# Autodesk Inventor assembly: RouveV4
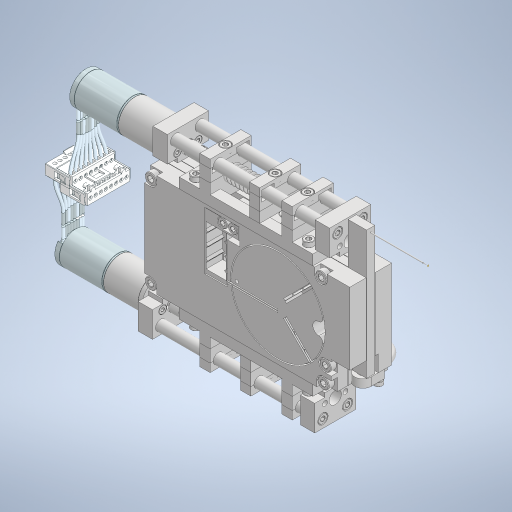
[picture p0: Inventor's stored thumbnail of the model, 512x512]
Saved by Autodesk Inventor 2023 (Build 270158000, 158)
## iProperties
Created: 2023-05-10
Part Number: RouveV4
Document SubType Name: Assembly
Designer: Nathann
Author: Nathann
## Documents named in this file (27)
- C:\Users\Nathann\OneDrive\ClawdDrive\Objet3D\IminaProbe\V4Roue\RouveV4.iam
- C:\Users\Nathann\OneDrive\ClawdDrive\Objet3D\IminaProbe\V4Roue\4145N198_Set Screw Precision Flexible Shaft Couplings.ipt
- C:\Users\Nathann\OneDrive\ClawdDrive\Objet3D\IminaProbe\V4Roue\283825_ec-max16_5w.ipt
- C:\Users\Nathann\OneDrive\ClawdDrive\Objet3D\IminaProbe\V4Roue\AngleScrewBlocActuator.ipt
- C:\Users\Nathann\OneDrive\ClawdDrive\Objet3D\IminaProbe\V4Roue\AxisLinear.ipt
- C:\Users\Nathann\OneDrive\ClawdDrive\Objet3D\IminaProbe\V4Roue\CapacitiveSensor.ipt
- C:\Users\Nathann\OneDrive\ClawdDrive\Objet3D\IminaProbe\V4Roue\MotorDifferentialMountingBracket.ipt
- C:\Users\Nathann\OneDrive\ClawdDrive\Objet3D\IminaProbe\V4Roue\MotorMountDifferential.ipt
- C:\Users\Nathann\OneDrive\ClawdDrive\Objet3D\IminaProbe\V4Roue\POMSliderAxis.ipt
- C:\Users\Nathann\OneDrive\ClawdDrive\Objet3D\IminaProbe\V4Roue\POMSliderMotor.ipt
- C:\Users\Nathann\OneDrive\ClawdDrive\Objet3D\IminaProbe\V4Roue\POMSliderMotorM25.ipt
- C:\Users\Nathann\OneDrive\ClawdDrive\Objet3D\IminaProbe\V4Roue\Probe.ipt
- C:\Users\Nathann\OneDrive\ClawdDrive\Objet3D\IminaProbe\V4Roue\RoueV3partA.ipt
- C:\Users\Nathann\OneDrive\ClawdDrive\Objet3D\IminaProbe\V4Roue\RoueV3PartB.ipt
- C:\Users\Nathann\OneDrive\ClawdDrive\Objet3D\IminaProbe\V4Roue\RoueV3PartC.ipt
- C:\Users\Nathann\OneDrive\ClawdDrive\Objet3D\IminaProbe\V4Roue\SliderFixtureM25.ipt
- C:\Users\Nathann\OneDrive\ClawdDrive\Objet3D\IminaProbe\V4Roue\Sprint.ipt
- C:\Users\Nathann\OneDrive\ClawdDrive\Objet3D\IminaProbe\V4Roue\GP16A_2-Stufig-110322.ipt
- C:\Users\Nathann\OneDrive\ClawdDrive\Objet3D\IminaProbe\V4Roue\Screw.ipt
- C:\Users\Nathann\ClawdDrive\Objet3D\IminaProbe\V3Roue\91292A009_18-8 Stainless Steel Socket Head Screw.ipt
- C:\Users\Nathann\ClawdDrive\Objet3D\IminaProbe\V3Roue\91292A832_18-8 Stainless Steel Socket Head Screw.ipt
- C:\Users\Nathann\ClawdDrive\Objet3D\IminaProbe\V3Roue\91828A113_18-8 Stainless Steel Hex Nut.ipt
- C:\Users\Nathann\ClawdDrive\Objet3D\IminaProbe\V3Roue\91828A211_18-8 Stainless Steel Hex Nut.ipt
- C:\Users\Nathann\OneDrive\ClawdDrive\Objet3D\IminaProbe\V4Roue\91292A012_18-8 Stainless Steel Socket Head Screw.ipt
- C:\Users\Nathann\OneDrive\ClawdDrive\Objet3D\IminaProbe\V4Roue\91292A114_18-8 Stainless Steel Socket Head Screw.ipt
- C:\Users\Nathann\OneDrive\ClawdDrive\Objet3D\IminaProbe\V4Roue\clinquantSpacer.ipt
- C:\Users\Nathann\OneDrive\ClawdDrive\Objet3D\IminaProbe\V4Roue\boundingBox.ipt
## Components (105 placed, 26 different names)
1. 4145N198_Set Screw Precision Flexible Shaft Couplings:1 — Insert:12, Insert:46
2. 283825_ec-max16_5w:1 — Insert:1, Mate:135
3. AngleScrewBlocActuator:1 — Insert:47, Insert:48
4. AxisLinear:1 — Mate:59, Mate:60, Insert:4, Insert:6, Mate:131
5. CapacitiveSensor:1 — Mate:2, Flush:7, Mate:3, Mate:4, Mate:37, Mate:38, Mate:39
6. MotorDifferentialMountingBracket:1 — Mate:47, Mate:48, Mate:49, Mate:50, Flush:12, Flush:13, Flush:14, Flush:15, Mate:51, Mate:52, Mate:53, Mate:54, Mate:55, Mate:56, Mate:57, Mate:58, Mate:73, Mate:75, Flush:25, Flush:26, Mate:118, Mate:119, Mate:120, Mate:121, Mate:122, Insert:31, Insert:32, Insert:33, Insert:34, Flush:42, Flush:45
7. MotorMountDifferential:1 — Mate:59, Mate:62, Mate:63, Mate:64, Mate:65, Mate:66, Mate:69, Mate:70, Insert:6, Insert:7, Insert:8, Insert:9, Insert:10, Insert:11
8. POMSliderAxis:1 — Flush:35, Flush:40, Mate:113, Mate:124, Insert:39
9. POMSliderMotor:1 — Flush:12, Flush:14, Mate:57, Flush:32, Mate:125, Mate:130
10. POMSliderMotorM25:1 — Flush:9, Flush:10, Mate:44, Mate:45, Mate:46, Flush:30, Flush:33, Mate:126, Flush:45
11. Probe:1 — Mate:1, Flush:8
12. RoueV3partA:1 — Flush:5, Flush:6, Mate:2, Flush:7, Mate:15, Mate:16, Mate:17, Mate:18, Mate:19, Mate:30, Mate:37, Angle:1, Mate:122, Mate:123
13. RoueV3PartB:1 — Flush:2, Flush:4, Mate:1, Flush:5, Flush:6, Mate:10, Mate:11, Mate:12, Mate:13, Mate:14, Mate:20, Mate:21, Mate:22, Mate:23, Mate:24, Mate:25, Mate:26, Mate:27, Mate:28, Mate:29, Flush:8
14. RoueV3PartC:1 — Flush:2, Flush:4, Mate:5, Mate:6, Mate:7, Mate:8, Mate:9, Mate:31, Mate:32, Mate:33, Mate:34, Mate:35, Mate:36, Flush:25, Flush:28, Flush:41, Mate:133, Mate:134, Insert:49, Insert:50, Mate:135
15. SliderFixtureM25:1 — Flush:9, Flush:10, Flush:11, Mate:45, Insert:2, Insert:3, Mate:73, Insert:13, Insert:14, Insert:47, Insert:48
16. Sprint:1 — Mate:75
17. GP16A_2-Stufig-110322:1 — Insert:1, Mate:63, Mate:66, Insert:11, Insert:45
18. Screw:1 — Insert:12
19. 91292A009_18-8 Stainless Steel Socket Head Screw:1 — Mate:113, Insert:39
20. 91292A832_18-8 Stainless Steel Socket Head Screw:2 — Mate:64, Insert:10
21. 91828A113_18-8 Stainless Steel Hex Nut:2 — Flush:11, Mate:44, Mate:46
22. 91828A211_18-8 Stainless Steel Hex Nut:1 — Mate:55, Mate:56
23. 91292A114_18-8 Stainless Steel Socket Head Screw:1 — Mate:5, Mate:33
24. 91292A832_18-8 Stainless Steel Socket Head Screw:3 — Mate:4, Mate:39
25. 91292A832_18-8 Stainless Steel Socket Head Screw:4 — Mate:3, Mate:38
26. 91292A114_18-8 Stainless Steel Socket Head Screw:2 — Mate:6, Mate:32
27. 91292A114_18-8 Stainless Steel Socket Head Screw:3 — Mate:8, Mate:34
28. 91292A114_18-8 Stainless Steel Socket Head Screw:4 — Mate:9, Mate:35
29. 91292A114_18-8 Stainless Steel Socket Head Screw:5 — Mate:7, Mate:36
30. clinquantSpacer:1 — Mate:13, Mate:26
31. clinquantSpacer:2 — Mate:12, Mate:25, Mate:31
32. clinquantSpacer:3 — Mate:14, Mate:28
33. clinquantSpacer:4 — Mate:10, Mate:27
34. clinquantSpacer:5 — Mate:11, Mate:29
35. clinquantSpacer:6 — Mate:18, Mate:22, Mate:30
36. clinquantSpacer:7 — Mate:19, Mate:23
37. clinquantSpacer:8 — Mate:17, Mate:20
38. clinquantSpacer:9 — Mate:16, Mate:24
39. clinquantSpacer:10 — Mate:15, Mate:21
40. MotorMountDifferential:2 — Mate:60, Mate:61, Mate:67, Mate:68, Insert:4, Insert:5, Mate:71, Mate:72, Flush:27
41. POMSliderAxis:2 — Mate:107, Flush:37, Flush:38, Mate:129, Insert:41
42. POMSliderAxis:3 — Mate:108, Mate:128, Insert:40, Flush:43, Flush:44
43. POMSliderMotor:2 — Flush:13, Flush:15, Mate:58, Flush:34, Mate:127
44. AxisLinear:2 — Mate:61, Mate:62, Insert:5
45. 91292A012_18-8 Stainless Steel Socket Head Screw:3 — Mate:69, Insert:8
46. 91292A009_18-8 Stainless Steel Socket Head Screw:2 — Insert:2
47. 91292A009_18-8 Stainless Steel Socket Head Screw:3 — Insert:3
48. 91292A009_18-8 Stainless Steel Socket Head Screw:4 — Mate:48, Mate:53
49. 91292A009_18-8 Stainless Steel Socket Head Screw:5 — Mate:50, Mate:51
50. 91292A009_18-8 Stainless Steel Socket Head Screw:6 — Mate:47, Mate:52
51. 91292A009_18-8 Stainless Steel Socket Head Screw:7 — Mate:49, Mate:54
52. 91292A012_18-8 Stainless Steel Socket Head Screw:4 — Mate:70, Insert:7
53. 91292A012_18-8 Stainless Steel Socket Head Screw:5 — Mate:67, Mate:72
54. 91292A012_18-8 Stainless Steel Socket Head Screw:6 — Mate:68, Mate:71
55. 91292A832_18-8 Stainless Steel Socket Head Screw:5 — Mate:65, Insert:9
56. 91292A012_18-8 Stainless Steel Socket Head Screw:7 — Insert:14
57. 91292A012_18-8 Stainless Steel Socket Head Screw:8 — Insert:13
58. 4145N198_Set Screw Precision Flexible Shaft Couplings:2 — Insert:45
59. MotorDifferentialMountingBracket:2 — Flush:27, Flush:28, Mate:114, Mate:115, Mate:116, Mate:117, Angle:1, Mate:123, Insert:35, Insert:36, Insert:37, Insert:38, Flush:42, Mate:132
60. POMSliderMotor:3 — Flush:35, Flush:40, Mate:124, Mate:131
61. POMSliderMotorM25:2 — Mate:128, Flush:43, Flush:44
62. SliderFixtureM25:2 — Mate:132
63. Screw:2
64. 91828A113_18-8 Stainless Steel Hex Nut:3
65. 91828A211_18-8 Stainless Steel Hex Nut:2
66. POMSliderMotor:4 — Flush:37, Flush:38, Mate:129
67. 91292A009_18-8 Stainless Steel Socket Head Screw:8
68. 91292A009_18-8 Stainless Steel Socket Head Screw:9
69. 91292A009_18-8 Stainless Steel Socket Head Screw:10
70. 91292A009_18-8 Stainless Steel Socket Head Screw:11
71. 91292A009_18-8 Stainless Steel Socket Head Screw:12
72. 91292A009_18-8 Stainless Steel Socket Head Screw:13
73. 91292A012_18-8 Stainless Steel Socket Head Screw:9
74. 91292A012_18-8 Stainless Steel Socket Head Screw:10
75. 283825_ec-max16_5w:2
76. AxisLinear:3 — Mate:130
77. MotorMountDifferential:3 — Flush:41
78. GP16A_2-Stufig-110322:2 — Insert:46
79. 91292A832_18-8 Stainless Steel Socket Head Screw:6
80. MotorMountDifferential:4 — Flush:26
81. AxisLinear:4
82. 91292A012_18-8 Stainless Steel Socket Head Screw:11
83. 91292A012_18-8 Stainless Steel Socket Head Screw:12
84. 91292A012_18-8 Stainless Steel Socket Head Screw:13
85. 91292A012_18-8 Stainless Steel Socket Head Screw:14
86. 91292A832_18-8 Stainless Steel Socket Head Screw:7
87. POMSliderAxis:4 — Mate:112, Flush:32, Mate:125, Insert:42
88. POMSliderAxis:5 — Mate:110, Flush:34, Mate:127, Insert:44
89. POMSliderAxis:6 — Mate:111, Flush:30, Flush:33, Mate:126, Insert:43
90. 91292A009_18-8 Stainless Steel Socket Head Screw:14 — Mate:108, Insert:40
91. 91292A009_18-8 Stainless Steel Socket Head Screw:15 — Mate:107, Insert:41
92. 91292A009_18-8 Stainless Steel Socket Head Screw:16 — Mate:112, Insert:42
93. 91292A009_18-8 Stainless Steel Socket Head Screw:17 — Mate:111, Insert:43
94. 91292A009_18-8 Stainless Steel Socket Head Screw:18 — Mate:110, Insert:44
95. 91292A012_18-8 Stainless Steel Socket Head Screw:15 — Mate:114, Insert:36
96. 91292A012_18-8 Stainless Steel Socket Head Screw:16 — Mate:115, Insert:37
97. 91292A012_18-8 Stainless Steel Socket Head Screw:17 — Mate:117, Insert:38
98. 91292A012_18-8 Stainless Steel Socket Head Screw:18 — Mate:116, Insert:35
99. 91292A012_18-8 Stainless Steel Socket Head Screw:19 — Mate:121, Insert:34
100. 91292A012_18-8 Stainless Steel Socket Head Screw:20 — Mate:120, Insert:33
101. 91292A012_18-8 Stainless Steel Socket Head Screw:21 — Mate:118, Insert:31
102. 91292A012_18-8 Stainless Steel Socket Head Screw:22 — Mate:119, Insert:32
103. 91292A012_18-8 Stainless Steel Socket Head Screw:23 — Mate:133, Insert:50
104. 91292A012_18-8 Stainless Steel Socket Head Screw:24 — Mate:134, Insert:49
105. boundingBox:1
## Relationships (214: Mate 128, Insert 48, Flush 37, Angle 1)
- Insert:1: 283825_ec-max16_5w:1 ↔ GP16A_2-Stufig-110322:1
- Flush:2: RoueV3PartB:1 ↔ RoueV3PartC:1
- Flush:4: RoueV3PartB:1 ↔ RoueV3PartC:1
- Mate:1: Probe:1 ↔ RoueV3PartB:1
- Flush:5: RoueV3partA:1 ↔ RoueV3PartB:1
- Flush:6: RoueV3partA:1 ↔ RoueV3PartB:1
- Mate:2: CapacitiveSensor:1 ↔ RoueV3partA:1
- Flush:7: CapacitiveSensor:1 ↔ RoueV3partA:1
- Mate:3: CapacitiveSensor:1 ↔ 91292A832_18-8 Stainless Steel Socket Head Screw:4
- Mate:4: CapacitiveSensor:1 ↔ 91292A832_18-8 Stainless Steel Socket Head Screw:3
- Mate:5: RoueV3PartC:1 ↔ 91292A114_18-8 Stainless Steel Socket Head Screw:1
- Mate:6: RoueV3PartC:1 ↔ 91292A114_18-8 Stainless Steel Socket Head Screw:2
- Mate:7: RoueV3PartC:1 ↔ 91292A114_18-8 Stainless Steel Socket Head Screw:5
- Mate:8: RoueV3PartC:1 ↔ 91292A114_18-8 Stainless Steel Socket Head Screw:3
- Mate:9: RoueV3PartC:1 ↔ 91292A114_18-8 Stainless Steel Socket Head Screw:4
- Mate:10: RoueV3PartB:1 ↔ clinquantSpacer:4
- Mate:11: RoueV3PartB:1 ↔ clinquantSpacer:5
- Mate:12: RoueV3PartB:1 ↔ clinquantSpacer:2
- Mate:13: RoueV3PartB:1 ↔ clinquantSpacer:1
- Mate:14: RoueV3PartB:1 ↔ clinquantSpacer:3
- Mate:15: RoueV3partA:1 ↔ clinquantSpacer:10
- Mate:16: RoueV3partA:1 ↔ clinquantSpacer:9
- Mate:17: RoueV3partA:1 ↔ clinquantSpacer:8
- Mate:18: RoueV3partA:1 ↔ clinquantSpacer:6
- Mate:19: RoueV3partA:1 ↔ clinquantSpacer:7
- Mate:20: RoueV3PartB:1 ↔ clinquantSpacer:8
- Mate:21: RoueV3PartB:1 ↔ clinquantSpacer:10
- Mate:22: RoueV3PartB:1 ↔ clinquantSpacer:6
- Mate:23: RoueV3PartB:1 ↔ clinquantSpacer:7
- Mate:24: RoueV3PartB:1 ↔ clinquantSpacer:9
- Mate:25: RoueV3PartB:1 ↔ clinquantSpacer:2
- Mate:26: RoueV3PartB:1 ↔ clinquantSpacer:1
- Mate:27: RoueV3PartB:1 ↔ clinquantSpacer:4
- Mate:28: RoueV3PartB:1 ↔ clinquantSpacer:3
- Mate:29: RoueV3PartB:1 ↔ clinquantSpacer:5
- Mate:30: RoueV3partA:1 ↔ clinquantSpacer:6
- Mate:31: RoueV3PartC:1 ↔ clinquantSpacer:2
- Mate:32: RoueV3PartC:1 ↔ 91292A114_18-8 Stainless Steel Socket Head Screw:2
- Mate:33: RoueV3PartC:1 ↔ 91292A114_18-8 Stainless Steel Socket Head Screw:1
- Mate:34: RoueV3PartC:1 ↔ 91292A114_18-8 Stainless Steel Socket Head Screw:3
- Mate:35: RoueV3PartC:1 ↔ 91292A114_18-8 Stainless Steel Socket Head Screw:4
- Mate:36: RoueV3PartC:1 ↔ 91292A114_18-8 Stainless Steel Socket Head Screw:5
- Flush:8 (-1 mm): Probe:1 ↔ RoueV3PartB:1
- Mate:37: CapacitiveSensor:1 ↔ RoueV3partA:1
- Mate:38: CapacitiveSensor:1 ↔ 91292A832_18-8 Stainless Steel Socket Head Screw:4
- Mate:39: CapacitiveSensor:1 ↔ 91292A832_18-8 Stainless Steel Socket Head Screw:3
- Flush:9: POMSliderMotorM25:1 ↔ SliderFixtureM25:1
- Flush:10: POMSliderMotorM25:1 ↔ SliderFixtureM25:1
- Flush:11 (-2 mm): SliderFixtureM25:1 ↔ 91828A113_18-8 Stainless Steel Hex Nut:2
- Mate:44: POMSliderMotorM25:1 ↔ 91828A113_18-8 Stainless Steel Hex Nut:2
- Mate:45: POMSliderMotorM25:1 ↔ SliderFixtureM25:1
- Mate:46: POMSliderMotorM25:1 ↔ 91828A113_18-8 Stainless Steel Hex Nut:2
- Insert:2: SliderFixtureM25:1 ↔ 91292A009_18-8 Stainless Steel Socket Head Screw:2
- Insert:3: SliderFixtureM25:1 ↔ 91292A009_18-8 Stainless Steel Socket Head Screw:3
- Mate:47: MotorDifferentialMountingBracket:1 ↔ 91292A009_18-8 Stainless Steel Socket Head Screw:6
- Mate:48: MotorDifferentialMountingBracket:1 ↔ 91292A009_18-8 Stainless Steel Socket Head Screw:4
- Mate:49: MotorDifferentialMountingBracket:1 ↔ 91292A009_18-8 Stainless Steel Socket Head Screw:7
- Mate:50: MotorDifferentialMountingBracket:1 ↔ 91292A009_18-8 Stainless Steel Socket Head Screw:5
- Flush:12: MotorDifferentialMountingBracket:1 ↔ POMSliderMotor:1
- Flush:13: MotorDifferentialMountingBracket:1 ↔ POMSliderMotor:2
- Flush:14: MotorDifferentialMountingBracket:1 ↔ POMSliderMotor:1
- Flush:15: MotorDifferentialMountingBracket:1 ↔ POMSliderMotor:2
- Mate:51: MotorDifferentialMountingBracket:1 ↔ 91292A009_18-8 Stainless Steel Socket Head Screw:5
- Mate:52: MotorDifferentialMountingBracket:1 ↔ 91292A009_18-8 Stainless Steel Socket Head Screw:6
- Mate:53: MotorDifferentialMountingBracket:1 ↔ 91292A009_18-8 Stainless Steel Socket Head Screw:4
- Mate:54: MotorDifferentialMountingBracket:1 ↔ 91292A009_18-8 Stainless Steel Socket Head Screw:7
- Mate:55: MotorDifferentialMountingBracket:1 ↔ 91828A211_18-8 Stainless Steel Hex Nut:1
- Mate:56: MotorDifferentialMountingBracket:1 ↔ 91828A211_18-8 Stainless Steel Hex Nut:1
- Mate:57: MotorDifferentialMountingBracket:1 ↔ POMSliderMotor:1
- Mate:58: MotorDifferentialMountingBracket:1 ↔ POMSliderMotor:2
- Mate:59: AxisLinear:1 ↔ MotorMountDifferential:1
- Mate:60: AxisLinear:1 ↔ MotorMountDifferential:2
- Mate:61: MotorMountDifferential:2 ↔ AxisLinear:2
- Mate:62: MotorMountDifferential:1 ↔ AxisLinear:2
- Mate:63: MotorMountDifferential:1 ↔ GP16A_2-Stufig-110322:1
- Mate:64: MotorMountDifferential:1 ↔ 91292A832_18-8 Stainless Steel Socket Head Screw:2
- Mate:65: MotorMountDifferential:1 ↔ 91292A832_18-8 Stainless Steel Socket Head Screw:5
- Mate:66: MotorMountDifferential:1 ↔ GP16A_2-Stufig-110322:1
- Mate:67: MotorMountDifferential:2 ↔ 91292A012_18-8 Stainless Steel Socket Head Screw:5
- Mate:68: MotorMountDifferential:2 ↔ 91292A012_18-8 Stainless Steel Socket Head Screw:6
- Mate:69: MotorMountDifferential:1 ↔ 91292A012_18-8 Stainless Steel Socket Head Screw:3
- Mate:70: MotorMountDifferential:1 ↔ 91292A012_18-8 Stainless Steel Socket Head Screw:4
- Insert:4: AxisLinear:1 ↔ MotorMountDifferential:2
- Insert:5: MotorMountDifferential:2 ↔ AxisLinear:2
- Insert:6: AxisLinear:1 ↔ MotorMountDifferential:1
- Insert:7: MotorMountDifferential:1 ↔ 91292A012_18-8 Stainless Steel Socket Head Screw:4
- Insert:8: MotorMountDifferential:1 ↔ 91292A012_18-8 Stainless Steel Socket Head Screw:3
- Insert:9: MotorMountDifferential:1 ↔ 91292A832_18-8 Stainless Steel Socket Head Screw:5
- Insert:10: MotorMountDifferential:1 ↔ 91292A832_18-8 Stainless Steel Socket Head Screw:2
- Mate:71: MotorMountDifferential:2 ↔ 91292A012_18-8 Stainless Steel Socket Head Screw:6
- Mate:72: MotorMountDifferential:2 ↔ 91292A012_18-8 Stainless Steel Socket Head Screw:5
- Insert:11: MotorMountDifferential:1 ↔ GP16A_2-Stufig-110322:1
- Mate:73: MotorDifferentialMountingBracket:1 ↔ SliderFixtureM25:1
- Insert:12 (-5 mm): 4145N198_Set Screw Precision Flexible Shaft Couplings:1 ↔ Screw:1
- Insert:13: SliderFixtureM25:1 ↔ 91292A012_18-8 Stainless Steel Socket Head Screw:8
- Insert:14: SliderFixtureM25:1 ↔ 91292A012_18-8 Stainless Steel Socket Head Screw:7
- Mate:75: MotorDifferentialMountingBracket:1 ↔ Sprint:1
- [Flush]: POMSliderMotorM25:2 ↔ SliderFixtureM25:2
- [Flush]: POMSliderMotorM25:2 ↔ SliderFixtureM25:2
- [Flush] (-2 mm): SliderFixtureM25:2 ↔ 91828A113_18-8 Stainless Steel Hex Nut:3
- [Mate]: POMSliderMotorM25:2 ↔ 91828A113_18-8 Stainless Steel Hex Nut:3
- [Mate]: POMSliderMotorM25:2 ↔ SliderFixtureM25:2
- [Mate]: POMSliderMotorM25:2 ↔ 91828A113_18-8 Stainless Steel Hex Nut:3
- [Insert]: SliderFixtureM25:2 ↔ 91292A009_18-8 Stainless Steel Socket Head Screw:8
- [Insert]: SliderFixtureM25:2 ↔ 91292A009_18-8 Stainless Steel Socket Head Screw:9
- [Mate]: MotorDifferentialMountingBracket:2 ↔ 91292A009_18-8 Stainless Steel Socket Head Screw:12
- [Mate]: MotorDifferentialMountingBracket:2 ↔ 91292A009_18-8 Stainless Steel Socket Head Screw:10
- [Mate]: MotorDifferentialMountingBracket:2 ↔ 91292A009_18-8 Stainless Steel Socket Head Screw:13
- [Mate]: MotorDifferentialMountingBracket:2 ↔ 91292A009_18-8 Stainless Steel Socket Head Screw:11
- [Flush]: MotorDifferentialMountingBracket:2 ↔ POMSliderMotor:3
- [Flush]: MotorDifferentialMountingBracket:2 ↔ POMSliderMotor:4
- [Flush]: MotorDifferentialMountingBracket:2 ↔ POMSliderMotor:3
- [Flush]: MotorDifferentialMountingBracket:2 ↔ POMSliderMotor:4
- [Mate]: MotorDifferentialMountingBracket:2 ↔ 91292A009_18-8 Stainless Steel Socket Head Screw:11
- [Mate]: MotorDifferentialMountingBracket:2 ↔ 91292A009_18-8 Stainless Steel Socket Head Screw:12
- [Mate]: MotorDifferentialMountingBracket:2 ↔ 91292A009_18-8 Stainless Steel Socket Head Screw:10
- [Mate]: MotorDifferentialMountingBracket:2 ↔ 91292A009_18-8 Stainless Steel Socket Head Screw:13
- [Mate]: MotorDifferentialMountingBracket:2 ↔ 91828A211_18-8 Stainless Steel Hex Nut:2
- [Mate]: MotorDifferentialMountingBracket:2 ↔ 91828A211_18-8 Stainless Steel Hex Nut:2
- [Mate]: MotorDifferentialMountingBracket:2 ↔ POMSliderMotor:3
- [Mate]: MotorDifferentialMountingBracket:2 ↔ POMSliderMotor:4
- [Mate]: MotorDifferentialMountingBracket:2 ↔ SliderFixtureM25:2
- [Insert] (-5 mm): 4145N198_Set Screw Precision Flexible Shaft Couplings:2 ↔ Screw:2
- [Insert]: SliderFixtureM25:2 ↔ 91292A012_18-8 Stainless Steel Socket Head Screw:10
- [Insert]: SliderFixtureM25:2 ↔ 91292A012_18-8 Stainless Steel Socket Head Screw:9
- [Insert]: 283825_ec-max16_5w:2 ↔ GP16A_2-Stufig-110322:2
- [Mate]: AxisLinear:3 ↔ MotorMountDifferential:3
- [Mate]: AxisLinear:3 ↔ MotorMountDifferential:4
- [Mate]: MotorMountDifferential:4 ↔ AxisLinear:4
- [Mate]: MotorMountDifferential:3 ↔ AxisLinear:4
- [Mate]: MotorMountDifferential:3 ↔ GP16A_2-Stufig-110322:2
- [Mate]: MotorMountDifferential:3 ↔ 91292A832_18-8 Stainless Steel Socket Head Screw:6
- [Mate]: MotorMountDifferential:3 ↔ 91292A832_18-8 Stainless Steel Socket Head Screw:7
- [Mate]: MotorMountDifferential:3 ↔ GP16A_2-Stufig-110322:2
- [Mate]: MotorMountDifferential:4 ↔ 91292A012_18-8 Stainless Steel Socket Head Screw:13
- [Mate]: MotorMountDifferential:4 ↔ 91292A012_18-8 Stainless Steel Socket Head Screw:14
- [Mate]: MotorMountDifferential:3 ↔ 91292A012_18-8 Stainless Steel Socket Head Screw:11
- [Mate]: MotorMountDifferential:3 ↔ 91292A012_18-8 Stainless Steel Socket Head Screw:12
- [Insert]: AxisLinear:3 ↔ MotorMountDifferential:4
- [Insert]: MotorMountDifferential:4 ↔ AxisLinear:4
- [Insert]: AxisLinear:3 ↔ MotorMountDifferential:3
- [Insert]: MotorMountDifferential:3 ↔ 91292A012_18-8 Stainless Steel Socket Head Screw:12
- [Insert]: MotorMountDifferential:3 ↔ 91292A012_18-8 Stainless Steel Socket Head Screw:11
- [Insert]: MotorMountDifferential:3 ↔ 91292A832_18-8 Stainless Steel Socket Head Screw:7
- [Insert]: MotorMountDifferential:3 ↔ 91292A832_18-8 Stainless Steel Socket Head Screw:6
- [Mate]: MotorMountDifferential:4 ↔ 91292A012_18-8 Stainless Steel Socket Head Screw:14
- [Mate]: MotorMountDifferential:4 ↔ 91292A012_18-8 Stainless Steel Socket Head Screw:13
- [Insert]: MotorMountDifferential:3 ↔ GP16A_2-Stufig-110322:2
- Flush:25: MotorDifferentialMountingBracket:1 ↔ RoueV3PartC:1
- Flush:26: MotorDifferentialMountingBracket:1 ↔ MotorMountDifferential:4
- Flush:27: MotorMountDifferential:2 ↔ MotorDifferentialMountingBracket:2
- Flush:28: RoueV3PartC:1 ↔ MotorDifferentialMountingBracket:2
- Mate:107: POMSliderAxis:2 ↔ 91292A009_18-8 Stainless Steel Socket Head Screw:15
- Mate:108: POMSliderAxis:3 ↔ 91292A009_18-8 Stainless Steel Socket Head Screw:14
- Mate:110: POMSliderAxis:5 ↔ 91292A009_18-8 Stainless Steel Socket Head Screw:18
- Mate:111: POMSliderAxis:6 ↔ 91292A009_18-8 Stainless Steel Socket Head Screw:17
- Mate:112: POMSliderAxis:4 ↔ 91292A009_18-8 Stainless Steel Socket Head Screw:16
- Flush:30: POMSliderMotorM25:1 ↔ POMSliderAxis:6
- Flush:32: POMSliderMotor:1 ↔ POMSliderAxis:4
- Flush:33: POMSliderMotorM25:1 ↔ POMSliderAxis:6
- Flush:34: POMSliderMotor:2 ↔ POMSliderAxis:5
- Flush:35: POMSliderAxis:1 ↔ POMSliderMotor:3
- Flush:37: POMSliderAxis:2 ↔ POMSliderMotor:4
- Flush:38: POMSliderAxis:2 ↔ POMSliderMotor:4
- Flush:40: POMSliderAxis:1 ↔ POMSliderMotor:3
- Mate:113: POMSliderAxis:1 ↔ 91292A009_18-8 Stainless Steel Socket Head Screw:1
- Mate:114: MotorDifferentialMountingBracket:2 ↔ 91292A012_18-8 Stainless Steel Socket Head Screw:15
- Mate:115: MotorDifferentialMountingBracket:2 ↔ 91292A012_18-8 Stainless Steel Socket Head Screw:16
- Mate:116: MotorDifferentialMountingBracket:2 ↔ 91292A012_18-8 Stainless Steel Socket Head Screw:18
- Mate:117: MotorDifferentialMountingBracket:2 ↔ 91292A012_18-8 Stainless Steel Socket Head Screw:17
- Mate:118: MotorDifferentialMountingBracket:1 ↔ 91292A012_18-8 Stainless Steel Socket Head Screw:21
- Mate:119: MotorDifferentialMountingBracket:1 ↔ 91292A012_18-8 Stainless Steel Socket Head Screw:22
- Mate:120: MotorDifferentialMountingBracket:1 ↔ 91292A012_18-8 Stainless Steel Socket Head Screw:20
- Mate:121: MotorDifferentialMountingBracket:1 ↔ 91292A012_18-8 Stainless Steel Socket Head Screw:19
- Flush:41: RoueV3PartC:1 ↔ MotorMountDifferential:3
- Angle:1 (0 deg): RoueV3partA:1 ↔ MotorDifferentialMountingBracket:2
- Mate:122: MotorDifferentialMountingBracket:1 ↔ RoueV3partA:1
- Mate:123: RoueV3partA:1 ↔ MotorDifferentialMountingBracket:2
- Insert:31: MotorDifferentialMountingBracket:1 ↔ 91292A012_18-8 Stainless Steel Socket Head Screw:21
- Insert:32: MotorDifferentialMountingBracket:1 ↔ 91292A012_18-8 Stainless Steel Socket Head Screw:22
- Insert:33: MotorDifferentialMountingBracket:1 ↔ 91292A012_18-8 Stainless Steel Socket Head Screw:20
- Insert:34: MotorDifferentialMountingBracket:1 ↔ 91292A012_18-8 Stainless Steel Socket Head Screw:19
- Insert:35: MotorDifferentialMountingBracket:2 ↔ 91292A012_18-8 Stainless Steel Socket Head Screw:18
- Insert:36: MotorDifferentialMountingBracket:2 ↔ 91292A012_18-8 Stainless Steel Socket Head Screw:15
- Insert:37: MotorDifferentialMountingBracket:2 ↔ 91292A012_18-8 Stainless Steel Socket Head Screw:16
- Insert:38: MotorDifferentialMountingBracket:2 ↔ 91292A012_18-8 Stainless Steel Socket Head Screw:17
- Flush:42: MotorDifferentialMountingBracket:1 ↔ MotorDifferentialMountingBracket:2
- Mate:124: POMSliderAxis:1 ↔ POMSliderMotor:3
- Mate:125: POMSliderMotor:1 ↔ POMSliderAxis:4
- Mate:126: POMSliderMotorM25:1 ↔ POMSliderAxis:6
- Mate:127: POMSliderMotor:2 ↔ POMSliderAxis:5
- Mate:128: POMSliderAxis:3 ↔ POMSliderMotorM25:2
- Mate:129: POMSliderAxis:2 ↔ POMSliderMotor:4
- Insert:39: POMSliderAxis:1 ↔ 91292A009_18-8 Stainless Steel Socket Head Screw:1
- Insert:40: POMSliderAxis:3 ↔ 91292A009_18-8 Stainless Steel Socket Head Screw:14
- Insert:41: POMSliderAxis:2 ↔ 91292A009_18-8 Stainless Steel Socket Head Screw:15
- Insert:42: POMSliderAxis:4 ↔ 91292A009_18-8 Stainless Steel Socket Head Screw:16
- Insert:43: POMSliderAxis:6 ↔ 91292A009_18-8 Stainless Steel Socket Head Screw:17
- Insert:44: POMSliderAxis:5 ↔ 91292A009_18-8 Stainless Steel Socket Head Screw:18
- Mate:130: POMSliderMotor:1 ↔ AxisLinear:3
- Mate:131: AxisLinear:1 ↔ POMSliderMotor:3
- Mate:132: MotorDifferentialMountingBracket:2 ↔ SliderFixtureM25:2
- Flush:43: POMSliderAxis:3 ↔ POMSliderMotorM25:2
- Flush:44: POMSliderAxis:3 ↔ POMSliderMotorM25:2
- Insert:45 (-4 mm): GP16A_2-Stufig-110322:1 ↔ 4145N198_Set Screw Precision Flexible Shaft Couplings:2
- Flush:45: MotorDifferentialMountingBracket:1 ↔ POMSliderMotorM25:1
- Insert:46 (-4 mm): 4145N198_Set Screw Precision Flexible Shaft Couplings:1 ↔ GP16A_2-Stufig-110322:2
- Insert:47: AngleScrewBlocActuator:1 ↔ SliderFixtureM25:1
- Insert:48: AngleScrewBlocActuator:1 ↔ SliderFixtureM25:1
- Mate:133: RoueV3PartC:1 ↔ 91292A012_18-8 Stainless Steel Socket Head Screw:23
- Mate:134: RoueV3PartC:1 ↔ 91292A012_18-8 Stainless Steel Socket Head Screw:24
- Insert:49: RoueV3PartC:1 ↔ 91292A012_18-8 Stainless Steel Socket Head Screw:24
- Insert:50: RoueV3PartC:1 ↔ 91292A012_18-8 Stainless Steel Socket Head Screw:23
- Mate:135 (-150 mm): 283825_ec-max16_5w:1 ↔ RoueV3PartC:1
## Named parameters: d109_d105 = 0 mm, d113_d52 = -2 mm, d114_d55 = 0 mm, d115_d56 = 0 mm, d116_d57 = 0 mm, d117_d60 = 0 mm, d118_d61 = 0 mm, d119_d62 = 0 mm, d120_d63 = 0 mm, d121_d64 = 0 mm, d122_d65 = 0 mm, d123_d100 = 0 mm, d126_d103 = -5 mm, d127_d104 = 0 mm, d128_d66 = 0 mm, d129_d67 = 0 mm, d130_d68 = 0 mm, d131_d69 = 0 mm, d132_d70 = 0 mm, d133_d71 = 0 mm, d134_d72 = 0 mm, d135_d73 = 0 mm, d136_d74 = 0 mm, d137_d75 = 0 mm, d138_d76 = 0 mm, d139_d77 = 0 mm, d140_d50 = 0 mm, d141_d51 = 0 mm, d142_d0 = 0 mm, d143_d81 = 0 mm, d144_d82 = 0 mm, d145_d83 = 0 mm, d146_d84 = 0 mm, d147_d85 = 0 mm, d148_d86 = 0 mm, d149_d87 = 0 mm, d150_d88 = 0 mm, d151_d89 = 0 mm, d152_d90 = 0 mm, d153_d91 = 0 mm, d154_d92 = 0 mm, d155_d93 = 0 mm, d156_d94 = 0 mm, d157_d95 = 0 mm, d158_d96 = 0 mm, d159_d97 = 0 mm, d160_d98 = 0 mm, d161_d99 = 0 mm, d162_d78 = 0 mm, d163_d79 = 0 mm, d164_d80 = 0 mm
